# Autodesk Inventor assembly: Main assembly
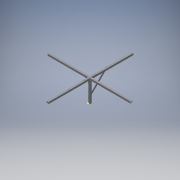
[picture p0: Inventor's stored thumbnail of the model, 180x180]
Saved by Autodesk Inventor 2017 (Build 210142000, 142)
## iProperties
Created: 2018-07-12
Part Number: Main assembly
Document SubType Name: Assembly
Designer: sinner
Author: sinner
## Documents named in this file (7)
- X:\Inventor files\Post\Main assembly.iam
- X:\Inventor files\Post\Lomg horizontal.ipt
- X:\Inventor files\Post\Short horizontal.ipt
- X:\Inventor files\Post\plate 1.ipt
- X:\Inventor files\Post\Vertical.ipt
- X:\Inventor files\Post\Bracket.ipt
- X:\Inventor files\Post\Long support flat.ipt
## Components (7 placed, 6 different names)
1. Lomg horizontal:1 — Flush:1, Mate:1, Flush:2, Mate:2, Flush:3, Flush:4, Mate:6, Mate:7, Flush:6
2. Short horizontal:1 — Mate:2, Flush:3, Flush:4, Mate:4, Mate:5, Flush:7, Angle:1
3. Short horizontal:2 — Flush:1, Mate:1, Flush:2, Mate:3
4. plate 1:1 — Mate:3, Mate:4, Mate:5
5. Vertical:1 — Mate:6, Mate:8, Flush:5, Flush:7, Mate:9, Mate:10
6. Bracket:1 — Mate:7, Mate:8, Flush:5, Flush:6
7. Long support flat:1 — Mate:9, Mate:10, Angle:1
## Relationships (18: Mate 10, Flush 7, Angle 1)
- Flush:1: Lomg horizontal:1 ↔ Short horizontal:2
- Mate:1: Lomg horizontal:1 ↔ Short horizontal:2
- Flush:2 (596.9 mm): Lomg horizontal:1 ↔ Short horizontal:2
- Mate:2: Lomg horizontal:1 ↔ Short horizontal:1
- Flush:3: Lomg horizontal:1 ↔ Short horizontal:1
- Flush:4 (-596.9 mm): Lomg horizontal:1 ↔ Short horizontal:1
- Mate:3: Short horizontal:2 ↔ plate 1:1
- Mate:4: Short horizontal:1 ↔ plate 1:1
- Mate:5: Short horizontal:1 ↔ plate 1:1
- Mate:6: Lomg horizontal:1 ↔ Vertical:1
- Mate:7: Lomg horizontal:1 ↔ Bracket:1
- Mate:8: Vertical:1 ↔ Bracket:1
- Flush:5: Vertical:1 ↔ Bracket:1
- Flush:6: Lomg horizontal:1 ↔ Bracket:1
- Flush:7: Short horizontal:1 ↔ Vertical:1
- Mate:9: Vertical:1 ↔ Long support flat:1
- Mate:10: Vertical:1 ↔ Long support flat:1
- Angle:1 (135 deg): Short horizontal:1 ↔ Long support flat:1
